# Autodesk Inventor assembly: PWTR-0136
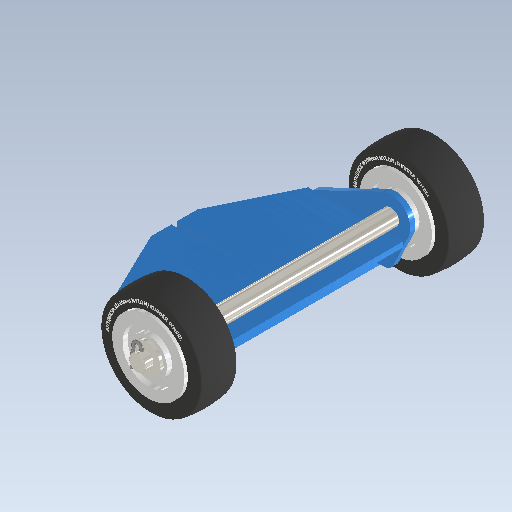
[picture p0: Inventor's stored thumbnail of the model, 512x512]
Saved by Autodesk Inventor 2021.1 (Build 251245010, 245A)
## iProperties
Created: 2020-09-03
Part Number: PWTR-0136
Document SubType Name: Assembly
Designer: alid
Author: alid
## Documents named in this file (6)
- C:\Users\peter\source\repos\InventorDA-FLC\Dataset\FY2021 Power Trowel\PWTR-0136.iam
- C:\Users\peter\source\repos\InventorDA-FLC\Dataset\FY2021 Power Trowel\PWTR-0135.ipt
- C:\Users\peter\source\repos\InventorDA-FLC\Dataset\FY2021 Power Trowel\PWTR-0137.ipt
- C:\Users\peter\source\repos\InventorDA-FLC\Dataset\FY2021 Power Trowel\PWTR-0138.ipt
- C:\Users\peter\source\repos\InventorDA-FLC\Dataset\FY2021 Power Trowel\PWTR-0139.ipt
- C:\Users\peter\source\repos\InventorDA-FLC\Dataset\FY2021 Power Trowel\PWTR-0114.ipt
## Components (6 placed, 6 different names)
1. Wheel Bracket — Insert:1, Insert:2, Insert:3, Insert:4
2. PWTR-0137:1 — Insert:1, Rigid:1
3. PWTR-0138:1 — Insert:2
4. Wheel — Insert:3
5. PWTR-0139:2 — Insert:4
6. PWTR-0114:1 — Rigid:1
## Relationships (5: Insert 4, WeldJoint 1)
- Insert:1 (40 mm): Wheel Bracket ↔ PWTR-0137:1
- Insert:2 (40 mm): Wheel Bracket ↔ PWTR-0138:1
- Insert:3: Wheel Bracket ↔ Wheel
- Insert:4: Wheel Bracket ↔ PWTR-0139:2
- Rigid:1 [WeldJoint]: PWTR-0137:1 ↔ PWTR-0114:1
